# Autodesk Inventor assembly: 어셈블리
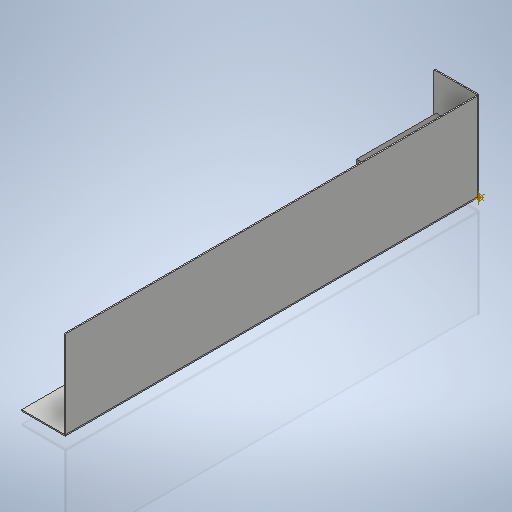
[picture p0: Inventor's stored thumbnail of the model, 512x512]
Saved by Autodesk Inventor 2025.1 (Build 291241000, 241)
## iProperties
Created: 2024-10-29
Part Number: 어셈블리
Document SubType Name: Assembly
Designer: gmsee
Mass: 1502.1 g
Surface Area: 8000.97 cm^2
Volume: 1502.1 cm^3
Density: 1 g/cm^3
Author: gmsee
## Documents named in this file (11)
- C:\Users\gmsee\Desktop\parts\가로로만\어셈블리.iam
- C:\Users\gmsee\Desktop\parts\가로로만\가로로만 옆판.ipt
- C:\Users\gmsee\Desktop\parts\가로로만\가로로만 윗판.ipt
- C:\Users\gmsee\Desktop\parts\가로로만\가로로만뒷판.ipt
- C:\Users\gmsee\Desktop\parts\기타파트\power supply.ipt
- C:\Users\gmsee\Desktop\parts\기타파트\만능기판.ipt
- C:\Users\gmsee\Desktop\parts\기타파트\비장애인.ipt
- C:\Users\gmsee\Desktop\parts\기타파트\장애인.ipt
- C:\Users\gmsee\Desktop\parts\기타파트\display.ipt
- C:\Users\gmsee\Desktop\parts\가로로만\가로로만.ipt
- C:\Users\gmsee\Desktop\parts\기타파트\스피커.ipt
## Components (13 placed, 10 different names)
1. 가로로만 옆판:1 — 메이트:3, 메이트:4, 메이트:7, 메이트:9, 메이트:10, 메이트:12, 메이트:13
2. 가로로만 윗판:1 — 메이트:7, 메이트:8, 메이트:14
3. 가로로만 옆판:2 — 메이트:5, 메이트:6, 메이트:21
4. 가로로만 윗판:2 — 메이트:2, 메이트:4, 메이트:6, 메이트:20
5. 가로로만뒷판:1 — 메이트:2, 메이트:3, 메이트:5, 메이트:8, 메이트:11, 메이트:15, 메이트:16, 메이트:17, 메이트:18, 메이트:19
6. power supply:1 — 메이트:11, 메이트:15, 메이트:18
7. 만능기판:1 — 메이트:16, 메이트:17, 메이트:19
8. 비장애인:1 — 메이트:24, 메이트:25
9. 장애인:1 — 메이트:22, 메이트:23
10. display:1 — 메이트:26, 메이트:27
11. display:2 — 메이트:28, 메이트:29
12. 가로로만:1 — 메이트:20, 메이트:21, 메이트:22, 메이트:23, 메이트:24, 메이트:25, 메이트:26, 메이트:27, 메이트:28, 메이트:29, 메이트:30, 메이트:31, 메이트:32
13. 스피커:1 — 메이트:30, 메이트:31, 메이트:32
## Relationships (31: Mate 31)
- 메이트:2 [Mate]: 가로로만 윗판:2 ↔ 가로로만뒷판:1
- 메이트:3 [Mate]: 가로로만 옆판:1 ↔ 가로로만뒷판:1
- 메이트:4 [Mate]: 가로로만 옆판:1 ↔ 가로로만 윗판:2
- 메이트:5 [Mate]: 가로로만 옆판:2 ↔ 가로로만뒷판:1
- 메이트:6 [Mate]: 가로로만 옆판:2 ↔ 가로로만 윗판:2
- 메이트:7 [Mate]: 가로로만 옆판:1 ↔ 가로로만 윗판:1
- 메이트:8 [Mate]: 가로로만 윗판:1 ↔ 가로로만뒷판:1
- 메이트:9 [Mate]: 가로로만 옆판:1
- 메이트:10 [Mate]: 가로로만 옆판:1
- 메이트:11 [Mate]: 가로로만뒷판:1 ↔ power supply:1
- 메이트:12 [Mate]: 가로로만 옆판:1
- 메이트:13 [Mate]: 가로로만 옆판:1
- 메이트:14 [Mate]: 가로로만 윗판:1
- 메이트:15 [Mate] (30 mm): 가로로만뒷판:1 ↔ power supply:1
- 메이트:16 [Mate]: 가로로만뒷판:1 ↔ 만능기판:1
- 메이트:17 [Mate] (20 mm): 가로로만뒷판:1 ↔ 만능기판:1
- 메이트:18 [Mate] (30 mm): 가로로만뒷판:1 ↔ power supply:1
- 메이트:19 [Mate] (100 mm): 가로로만뒷판:1 ↔ 만능기판:1
- 메이트:20 [Mate]: 가로로만 윗판:2 ↔ 가로로만:1
- 메이트:21 [Mate]: 가로로만 옆판:2 ↔ 가로로만:1
- 메이트:22 [Mate]: 장애인:1 ↔ 가로로만:1
- 메이트:23 [Mate]: 장애인:1 ↔ 가로로만:1
- 메이트:24 [Mate]: 비장애인:1 ↔ 가로로만:1
- 메이트:25 [Mate]: 비장애인:1 ↔ 가로로만:1
- 메이트:26 [Mate]: display:1 ↔ 가로로만:1
- 메이트:27 [Mate]: display:1 ↔ 가로로만:1
- 메이트:28 [Mate]: display:2 ↔ 가로로만:1
- 메이트:29 [Mate]: display:2 ↔ 가로로만:1
- 메이트:30 [Mate]: 가로로만:1 ↔ 스피커:1
- 메이트:31 [Mate]: 가로로만:1 ↔ 스피커:1
- 메이트:32 [Mate]: 가로로만:1 ↔ 스피커:1
